# Autodesk Inventor assembly: FreeBOT_simplified_clean
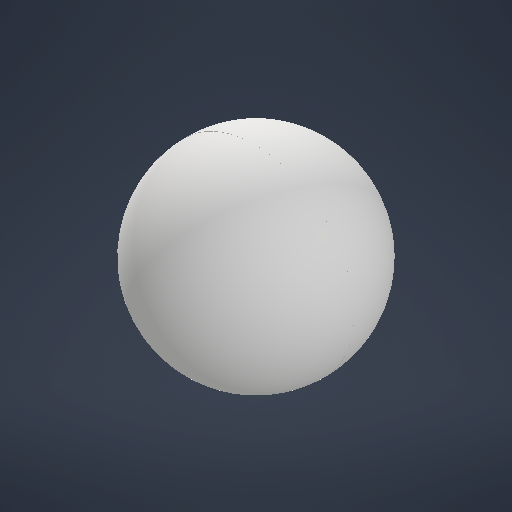
[picture p0: Inventor's stored thumbnail of the model, 512x512]
Saved by Autodesk Inventor 2027 (Build 310192060, 192F)
## iProperties
Created: 1601-01-02
Part Number: FreeBOT_simplified_clean
Document SubType Name: Assembly
Designer: loren
Part Number: GM12-N20VA-Motor
Sending System: SOLIDWORKS 2018
Last Saved Date: 2022-07-07
Author: loren
## Documents named in this file (20)
- C:\Users\loren\Desktop\Tesi Magistrale\CAD\FreeBOT\FreeBOT_simplified_clean.iam
- C:\Users\loren\Downloads\n20-14.snapshot.1\N20后侧输出轴\GM12-N20VA-Motor\M057-8Y01A.iam
- C:\Users\loren\Downloads\n20-14.snapshot.1\N20后侧输出轴\GM12-N20VA-Motor\减速机支架.ipt
- C:\Users\loren\Downloads\n20-14.snapshot.1\N20后侧输出轴\GM12-N20VA-Motor\十字沉头螺丝.ipt
- C:\Users\loren\Downloads\n20-14.snapshot.1\N20后侧输出轴\GM12-N20VA-Motor\Engrenagem reta28-D.ipt
- C:\Users\loren\Desktop\Tesi Magistrale\CAD\FreeBOT\chassis.ipt
- C:\Users\loren\Desktop\Tesi Magistrale\CAD\FreeBOT\chassis3.ipt
- C:\Users\loren\Desktop\Tesi Magistrale\CAD\FreeBOT\Pololu-Wheel-32x7mm.iam
- C:\Users\loren\Desktop\Tesi Magistrale\CAD\FreeBOT\tronco_ruote.ipt
- C:\Users\loren\Desktop\Tesi Magistrale\CAD\FreeBOT\tronco_ruota_2.ipt
- C:\Users\loren\Desktop\Tesi Magistrale\CAD\FreeBOT\chassis 2.ipt
- C:\Users\loren\Desktop\Tesi Magistrale\CAD\FreeBOT\tronco_ruota3.ipt
- C:\Users\loren\Desktop\Tesi Magistrale\CAD\FreeBOT\magnete.ipt
- C:\Users\loren\Desktop\Tesi Magistrale\CAD\FreeBOT\guscio sferico B.ipt.iam
- C:\Users\loren\Downloads\pololu-ball-caster-with-3-8-plastic-metal-ball-1.snapshot.3\Rueda loca\Pololu Ball Caster\base.ipt
- C:\Users\loren\Downloads\pololu-ball-caster-with-3-8-plastic-metal-ball-1.snapshot.3\Rueda loca\Pololu Ball Caster\ball.ipt
- C:\Users\loren\Desktop\Tesi Magistrale\CAD\FreeBOT\telaio per casters.ipt
- C:\Users\loren\Desktop\Tesi Magistrale\CAD\FreeBOT\base_telaio_casters.ipt
- C:\Users\loren\Desktop\Tesi Magistrale\CAD\FreeBOT\guscio sferico_A.iam
- guscio sferico B.ipt
## Components (32 placed, 21 different names)
1. M057-8Y01A-1 [sub-assembly] — Rigid:1, Mate:4, Mate:5, Mate:6
2. 减速机支架-1 — Rigid:1, Rigid:3, Rotational:7, Mate:7, Mate:13
3. 十字沉头螺丝-1 — Rigid:3
4. Engrenagem reta28-D-1 — Rotational:7, Mate:15, Rigid:7
5. chassis:1 — Mate:1, Mate:2, Mate:3, Mate:4, Mate:5, Mate:8, Mate:9, Mate:10, Mate:11, Rigid:19, Rigid:26, Rigid:27, Rigid:28, Rigid:29
6. chassis3:1 — Mate:1, Mate:2, Mate:3, Mate:6, Mate:7, Mate:13
7. M057-8Y01A:2 [sub-assembly] — Mate:10, Mate:11, Mate:12
8. 减速机支架:2 — Mate:14
9. Engrenagem reta28-D:2 — Mate:16, Rigid:25
10. chassis3:2 — Mate:8, Mate:9, Mate:12, Mate:14
11. Pololu-Wheel-32x7mm:1 [sub-assembly] — Rigid:17, Rigid:18
12. tronco_ruote:1 — Mate:15, Rigid:7, Rigid:16
13. tronco_ruota_2:1 — Rigid:16, Rigid:17
14. tronco_ruota_2:2 — Rigid:18
15. chassis 2:1 — Rigid:19, Rigid:20
16. tronco_ruota3:1 — Rigid:20
17. Pololu-Wheel-32x7mm:2 [sub-assembly]
18. tronco_ruote:2 — Mate:16, Rigid:25
19. tronco_ruota_2:3
20. tronco_ruota_2:4
21. chassis 2:2 — Rigid:26
22. tronco_ruota3:2
23. magnete:1 — Rigid:27
24. guscio sferico B.ipt:1 [sub-assembly] — Mate:18
25. base:1 — Ball:1, Rotational:15, Rotational:16
26. ball:1 — Ball:1
27. telaio per casters:1 — Rotational:15, Rotational:16, Mate:17, Rotational:17, Rotational:18, Rotational:19, Rotational:20, Rigid:30
28. base:2 — Mate:17, Rotational:17, Rotational:18, Rotational:19, Rotational:20
29. ball:2
30. base_telaio_casters:1 — Rigid:28
31. base_telaio_casters:2 — Rigid:29, Rigid:30
32. guscio sferico_A:1 [sub-assembly] — Mate:18
## Relationships (47: WeldJoint 19, Mate 18, RevoluteJoint 8, BallJoint 2)
- Rigid:1 [WeldJoint]: M057-8Y01A-1 ↔ 减速机支架-1
- Rigid:3 [WeldJoint]: 减速机支架-1 ↔ 十字沉头螺丝-1
- Rotational:7 [RevoluteJoint]: 减速机支架-1 ↔ Engrenagem reta28-D-1
- Mate:1: chassis:1 ↔ chassis3:1
- Mate:2: chassis:1 ↔ chassis3:1
- Mate:3: chassis:1 ↔ chassis3:1
- Mate:4: M057-8Y01A-1 ↔ chassis:1
- Mate:5: M057-8Y01A-1 ↔ chassis:1
- Mate:6: M057-8Y01A-1 ↔ chassis3:1
- Mate:7: 减速机支架-1 ↔ chassis3:1
- [WeldJoint]: M057-8Y01A:2 ↔ 减速机支架:2
- [RevoluteJoint]: 减速机支架:2 ↔ Engrenagem reta28-D:2
- Mate:8: chassis:1 ↔ chassis3:2
- Mate:9: chassis:1 ↔ chassis3:2
- Mate:10: chassis:1 ↔ M057-8Y01A:2
- Mate:11: chassis:1 ↔ M057-8Y01A:2
- Mate:12: M057-8Y01A:2 ↔ chassis3:2
- Mate:13: 减速机支架-1 ↔ chassis3:1
- Mate:14: 减速机支架:2 ↔ chassis3:2
- Mate:15: Engrenagem reta28-D-1 ↔ tronco_ruote:1
- Rigid:7 [WeldJoint]: Engrenagem reta28-D-1 ↔ tronco_ruote:1
- Rigid:16 [WeldJoint]: tronco_ruote:1 ↔ tronco_ruota_2:1
- Rigid:17 [WeldJoint]: Pololu-Wheel-32x7mm:1 ↔ tronco_ruota_2:1
- Rigid:18 [WeldJoint]: Pololu-Wheel-32x7mm:1 ↔ tronco_ruota_2:2
- Rigid:19 [WeldJoint]: chassis:1 ↔ chassis 2:1
- Rigid:20 [WeldJoint]: chassis 2:1 ↔ tronco_ruota3:1
- [WeldJoint]: tronco_ruote:2 ↔ tronco_ruota_2:3
- [WeldJoint]: Pololu-Wheel-32x7mm:2 ↔ tronco_ruota_2:3
- [WeldJoint]: Pololu-Wheel-32x7mm:2 ↔ tronco_ruota_2:4
- [WeldJoint]: chassis 2:2 ↔ tronco_ruota3:2
- Mate:16: Engrenagem reta28-D:2 ↔ tronco_ruote:2
- Rigid:25 [WeldJoint]: Engrenagem reta28-D:2 ↔ tronco_ruote:2
- Rigid:26 [WeldJoint]: chassis:1 ↔ chassis 2:2
- Rigid:27 [WeldJoint]: chassis:1 ↔ magnete:1
- Ball:1: base:1 ↔ ball:1
- Rotational:15 [RevoluteJoint]: base:1 ↔ telaio per casters:1
- Rotational:16 [RevoluteJoint]: base:1 ↔ telaio per casters:1
- [BallJoint]: base:2 ↔ ball:2
- Mate:17: telaio per casters:1 ↔ base:2
- Rotational:17 [RevoluteJoint]: telaio per casters:1 ↔ base:2
- Rotational:18 [RevoluteJoint]: telaio per casters:1 ↔ base:2
- Rotational:19 [RevoluteJoint]: telaio per casters:1 ↔ base:2
- Rotational:20 [RevoluteJoint]: telaio per casters:1 ↔ base:2
- Rigid:28 [WeldJoint]: chassis:1 ↔ base_telaio_casters:1
- Rigid:29 [WeldJoint]: chassis:1 ↔ base_telaio_casters:2
- Rigid:30 [WeldJoint]: telaio per casters:1 ↔ base_telaio_casters:2
- Mate:18: guscio sferico B.ipt:1 ↔ guscio sferico_A:1
## Named parameters: d38_d0 = 0 mm, d53_d27 = 0 mm, d54_d28 = -1.315162 deg, d76_d75 = 0 mm, d77_d66 = 0 mm, d78_d67 = 7.193377 deg, d79_d70 = 0 mm, d80_d71 = 0 mm
